# Autodesk Inventor assembly: frame assembly 6
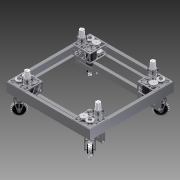
[picture p0: Inventor's stored thumbnail of the model, 180x180]
Saved by Autodesk Inventor 2012 (Build 160160000, 160)
## iProperties
Created: 2013-07-20
Part Number: frame assembly 6
Document SubType Name: Assembly
Designer: Bryce
Author: Bryce
## Documents named in this file (5)
- C:\Users\Bryce\Dropbox\Inventor Design Project Files\Independent Swerves\Inventor 2012\frame assembly 6.iam
- C:\Users\Bryce\Dropbox\Inventor Design Project Files\Independent Swerves\Inventor 2012\frame U 1 by 3.ipt
- C:\Users\Bryce\Dropbox\Inventor Design Project Files\Independent Swerves\Inventor 2012\FULL SWERVE DRIVE ASSEMBLY!  2!.iam
- C:\Users\Bryce\Dropbox\Inventor Design Project Files\Independent Swerves\Inventor 2012\frame undermount 1 by 3.ipt
- C:\Users\Bryce\Dropbox\Inventor Design Project Files\Independent Swerves\Inventor 2012\frame box 1 by 2.ipt
## Components (14 placed, 4 different names)
1. frame U 1 by 3:1 — Mate:1, Mate:4, Mate:5, Flush:1, Flush:2, Mate:7, Mate:10, Mate:11, Flush:7, Mate:21
2. frame U 1 by 3:2 — Mate:1, Mate:2, Flush:1, Flush:3, Mate:6, Mate:8, Mate:16, Mate:17
3. frame U 1 by 3:3 — Mate:2, Mate:3, Flush:3, Mate:14, Mate:15, Flush:4, Mate:18, Mate:24, Flush:13
4. frame U 1 by 3:4 — Mate:3, Mate:4, Mate:5, Flush:2, Mate:9, Mate:12, Mate:13
5. FULL SWERVE DRIVE ASSEMBLY!  2!:1 [sub-assembly] — Mate:6, Mate:7, Mate:8
6. FULL SWERVE DRIVE ASSEMBLY!  2!:2 [sub-assembly] — Mate:9, Mate:10, Mate:11
7. FULL SWERVE DRIVE ASSEMBLY!  2!:3 [sub-assembly] — Mate:12, Mate:13, Mate:14, Mate:19
8. FULL SWERVE DRIVE ASSEMBLY!  2!:4 [sub-assembly] — Mate:15, Mate:16, Mate:17, Mate:25
9. frame undermount 1 by 3:1 — Flush:4, Mate:18, Mate:19, Mate:20, Flush:5, Flush:6
10. frame undermount 1 by 3:2 — Flush:7, Mate:21, Flush:8
11. frame undermount 1 by 3:3 — Mate:23, Flush:11, Flush:12, Mate:24, Flush:13, Mate:25
12. frame undermount 1 by 3:4 — Mate:22, Flush:9, Flush:10
13. frame box 1 by 2:1 — Mate:20, Flush:5, Flush:6, Flush:8
14. frame box 1 by 2:2 — Mate:22, Flush:9, Flush:10, Mate:23, Flush:11, Flush:12
## Relationships (38: Mate 25, Flush 13)
- Mate:1: frame U 1 by 3:1 ↔ frame U 1 by 3:2
- Mate:2: frame U 1 by 3:2 ↔ frame U 1 by 3:3
- Mate:3: frame U 1 by 3:3 ↔ frame U 1 by 3:4
- Mate:4: frame U 1 by 3:1 ↔ frame U 1 by 3:4
- Mate:5: frame U 1 by 3:1 ↔ frame U 1 by 3:4
- Flush:1: frame U 1 by 3:1 ↔ frame U 1 by 3:2
- Flush:2: frame U 1 by 3:1 ↔ frame U 1 by 3:4
- Flush:3: frame U 1 by 3:2 ↔ frame U 1 by 3:3
- Mate:6: frame U 1 by 3:2 ↔ FULL SWERVE DRIVE ASSEMBLY!  2!:1
- Mate:7: frame U 1 by 3:1 ↔ FULL SWERVE DRIVE ASSEMBLY!  2!:1
- Mate:8: frame U 1 by 3:2 ↔ FULL SWERVE DRIVE ASSEMBLY!  2!:1
- Mate:9: frame U 1 by 3:4 ↔ FULL SWERVE DRIVE ASSEMBLY!  2!:2
- Mate:10: frame U 1 by 3:1 ↔ FULL SWERVE DRIVE ASSEMBLY!  2!:2
- Mate:11: frame U 1 by 3:1 ↔ FULL SWERVE DRIVE ASSEMBLY!  2!:2
- Mate:12: frame U 1 by 3:4 ↔ FULL SWERVE DRIVE ASSEMBLY!  2!:3
- Mate:13: frame U 1 by 3:4 ↔ FULL SWERVE DRIVE ASSEMBLY!  2!:3
- Mate:14: frame U 1 by 3:3 ↔ FULL SWERVE DRIVE ASSEMBLY!  2!:3
- Mate:15: frame U 1 by 3:3 ↔ FULL SWERVE DRIVE ASSEMBLY!  2!:4
- Mate:16: frame U 1 by 3:2 ↔ FULL SWERVE DRIVE ASSEMBLY!  2!:4
- Mate:17: frame U 1 by 3:2 ↔ FULL SWERVE DRIVE ASSEMBLY!  2!:4
- Flush:4: frame U 1 by 3:3 ↔ frame undermount 1 by 3:1
- Mate:18: frame U 1 by 3:3 ↔ frame undermount 1 by 3:1
- Mate:19 (-50.8 mm): FULL SWERVE DRIVE ASSEMBLY!  2!:3 ↔ frame undermount 1 by 3:1
- Mate:20: frame undermount 1 by 3:1 ↔ frame box 1 by 2:1
- Flush:5: frame undermount 1 by 3:1 ↔ frame box 1 by 2:1
- Flush:6: frame undermount 1 by 3:1 ↔ frame box 1 by 2:1
- Flush:7: frame U 1 by 3:1 ↔ frame undermount 1 by 3:2
- Mate:21: frame U 1 by 3:1 ↔ frame undermount 1 by 3:2
- Flush:8: frame undermount 1 by 3:2 ↔ frame box 1 by 2:1
- Mate:22: frame undermount 1 by 3:4 ↔ frame box 1 by 2:2
- Flush:9: frame undermount 1 by 3:4 ↔ frame box 1 by 2:2
- Flush:10: frame undermount 1 by 3:4 ↔ frame box 1 by 2:2
- Mate:23: frame undermount 1 by 3:3 ↔ frame box 1 by 2:2
- Flush:11: frame undermount 1 by 3:3 ↔ frame box 1 by 2:2
- Flush:12: frame undermount 1 by 3:3 ↔ frame box 1 by 2:2
- Mate:24: frame U 1 by 3:3 ↔ frame undermount 1 by 3:3
- Flush:13: frame U 1 by 3:3 ↔ frame undermount 1 by 3:3
- Mate:25 (-50.8 mm): FULL SWERVE DRIVE ASSEMBLY!  2!:4 ↔ frame undermount 1 by 3:3
